# Autodesk Inventor assembly: КВ33.044.200
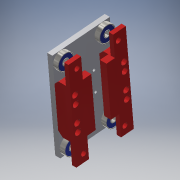
[picture p0: Inventor's stored thumbnail of the model, 180x180]
Saved by Autodesk Inventor 2019 (Build 230136000, 136)
## iProperties
Created: 2019-07-15
Part Number: КВ33.044.200
Material: Типовые
Document SubType Name: Assembly
Designer: Петров Иван
Description: Каретка оси Х
Author: Петров Иван
## Documents named in this file (4)
- C:\Users\user\Documents\Kvantoriada2019\optimal_gripper\hardware\КВ33.044.200 - Каретка оси Х.iam
- C:\Users\user\Documents\Kvantoriada2019\optimal_gripper\hardware\Стандартные изделия\Подшипник 626Z.ipt
- C:\Users\user\Documents\Kvantoriada2019\optimal_gripper\hardware\КВ33.044.202 - Фиксатор каретки.ipt
- C:\Users\user\Documents\Kvantoriada2019\optimal_gripper\hardware\КВ33.044.201 - Щека каретки.ipt
## Components (7 placed, 3 different names)
1. КВ33.044.201 - Щека каретки:1 — Жесткий:1, Жесткий:2, Совмещение:1, Совмещение:2, Совмещение:3, Совмещение:4, Совмещение:5, Совмещение:6, Совмещение:7, Совмещение:8
2. Подшипник 626Z:1 — Совмещение:3, Совмещение:4
3. Подшипник 626Z:2 — Совмещение:1, Совмещение:2
4. Подшипник 626Z:3 — Совмещение:7, Совмещение:8
5. Подшипник 626Z:4 — Совмещение:5, Совмещение:6
6. КВ33.044.202 - Фиксатор каретки:1 — Жесткий:1
7. КВ33.044.202 - Фиксатор каретки:2 — Жесткий:2
## Relationships (10: Mate 8, WeldJoint 2)
- Жесткий:1 [WeldJoint]: КВ33.044.201 - Щека каретки:1 ↔ КВ33.044.202 - Фиксатор каретки:1
- Жесткий:2 [WeldJoint]: КВ33.044.201 - Щека каретки:1 ↔ КВ33.044.202 - Фиксатор каретки:2
- Совмещение:1 [Mate]: КВ33.044.201 - Щека каретки:1 ↔ Подшипник 626Z:2
- Совмещение:2 [Mate]: КВ33.044.201 - Щека каретки:1 ↔ Подшипник 626Z:2
- Совмещение:3 [Mate]: КВ33.044.201 - Щека каретки:1 ↔ Подшипник 626Z:1
- Совмещение:4 [Mate]: КВ33.044.201 - Щека каретки:1 ↔ Подшипник 626Z:1
- Совмещение:5 [Mate]: КВ33.044.201 - Щека каретки:1 ↔ Подшипник 626Z:4
- Совмещение:6 [Mate]: КВ33.044.201 - Щека каретки:1 ↔ Подшипник 626Z:4
- Совмещение:7 [Mate]: КВ33.044.201 - Щека каретки:1 ↔ Подшипник 626Z:3
- Совмещение:8 [Mate]: КВ33.044.201 - Щека каретки:1 ↔ Подшипник 626Z:3
